# Autodesk Inventor assembly: Robot
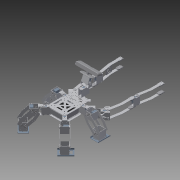
[picture p0: Inventor's stored thumbnail of the model, 180x180]
Saved by Autodesk Inventor 2013 (Build 170138000, 138)
## iProperties
Created: 2014-05-11
Part Number: Robot
Document SubType Name: Assembly
Designer: andou
Mass: 3393.74 g
Surface Area: 11048.5 cm^2
Volume: 1954.38 cm^3
Density: 1.73648 g/cm^3
Author: andou
## Documents named in this file (8)
- C:\Users\andou\Documents\Inventor\RoboticsProject\project_4\Robot\Robot.iam
- C:\Users\andou\Documents\Inventor\RoboticsProject\project_4\Robot\Body\Main Plate.ipt
- C:\Users\andou\Documents\Inventor\RoboticsProject\project_4\Robot\Leg\Left_Leg\Left Leg.iam
- C:\Users\andou\Documents\Inventor\RoboticsProject\project_4\Robot\Leg\Right_Leg\Right Leg.iam
- C:\Users\andou\Documents\Inventor\RoboticsProject\project_4\Robot\Head\Head.iam
- C:\Users\andou\Documents\Inventor\RoboticsProject\project_4\Robot\Arm\Left_Arm\Left_Arm.iam
- C:\Users\andou\Documents\Inventor\RoboticsProject\project_4\Robot\Body\BRIX.ipt
- C:\Users\andou\Documents\Inventor\RoboticsProject\project_4\Robot\Arm\Right_Arm\Right_Arm.iam
## Components (10 placed, 7 different names)
1. Main Plate:1 — 挿入:13, 挿入:14, 挿入:15, 挿入:16, 挿入:17, 挿入:18, 挿入:19, 挿入:20, 挿入:37, 挿入:38, 挿入:39, 挿入:40, 挿入:41, 挿入:42
2. Left Leg:1 [sub-assembly] — 挿入:13, 挿入:19
3. Left Leg:2 [sub-assembly] — 挿入:14, 挿入:20, 挿入:46
4. Right Leg:1 [sub-assembly] — 挿入:16, 挿入:17
5. Right Leg:2 [sub-assembly] — 挿入:15, 挿入:18, 挿入:45
6. Head:1 [sub-assembly] — 挿入:43, 挿入:44
7. Left_Arm:1 [sub-assembly] — 挿入:39, 挿入:40
8. BRIX:1 — 挿入:37, 挿入:38
9. Right_Arm:1 [sub-assembly] — 挿入:41, 挿入:42
10. Main Plate:2 — 挿入:43, 挿入:44, 挿入:45, 挿入:46
## Relationships (18: Insert 18)
- 挿入:13 [Insert]: Main Plate:1 ↔ Left Leg:1
- 挿入:14 [Insert]: Main Plate:1 ↔ Left Leg:2
- 挿入:15 [Insert]: Main Plate:1 ↔ Right Leg:2
- 挿入:16 [Insert]: Main Plate:1 ↔ Right Leg:1
- 挿入:17 [Insert]: Main Plate:1 ↔ Right Leg:1
- 挿入:18 [Insert]: Main Plate:1 ↔ Right Leg:2
- 挿入:19 [Insert]: Main Plate:1 ↔ Left Leg:1
- 挿入:20 [Insert]: Main Plate:1 ↔ Left Leg:2
- 挿入:37 [Insert]: Main Plate:1 ↔ BRIX:1
- 挿入:38 [Insert]: Main Plate:1 ↔ BRIX:1
- 挿入:39 [Insert]: Main Plate:1 ↔ Left_Arm:1
- 挿入:40 [Insert]: Main Plate:1 ↔ Left_Arm:1
- 挿入:41 [Insert]: Main Plate:1 ↔ Right_Arm:1
- 挿入:42 [Insert]: Main Plate:1 ↔ Right_Arm:1
- 挿入:43 [Insert]: Head:1 ↔ Main Plate:2
- 挿入:44 [Insert]: Head:1 ↔ Main Plate:2
- 挿入:45 [Insert]: Right Leg:2 ↔ Main Plate:2
- 挿入:46 [Insert]: Left Leg:2 ↔ Main Plate:2
